# Autodesk Inventor assembly: Second Extension of Base
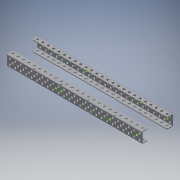
[picture p0: Inventor's stored thumbnail of the model, 180x180]
Saved by Autodesk Inventor 2018 (Build 220112000, 112)
## iProperties
Created: 2017-06-28
Part Number: Second Extension of Base
Document SubType Name: Assembly
Designer: James
Author: James
## Documents named in this file (2)
- C:\Users\James\Desktop\EE REU\Hardware\Vex Arm\Second Extension of Base.iam
- C:\Users\James\Desktop\EE REU\Hardware\Vex Arm\Vex Parts\C_Channel.ipt
## Components (2 placed, 1 different names)
1. C_Channel:1 — Flush:1, Mate:1, Flush:2
2. C_Channel:2 — Flush:1, Mate:1, Flush:2
## Relationships (3: Flush 2, Mate 1)
- Flush:1: C_Channel:1 ↔ C_Channel:2
- Mate:1 (70 mm): C_Channel:1 ↔ C_Channel:2
- Flush:2: C_Channel:1 ↔ C_Channel:2
